# Autodesk Inventor assembly: Ring Stand Clamp
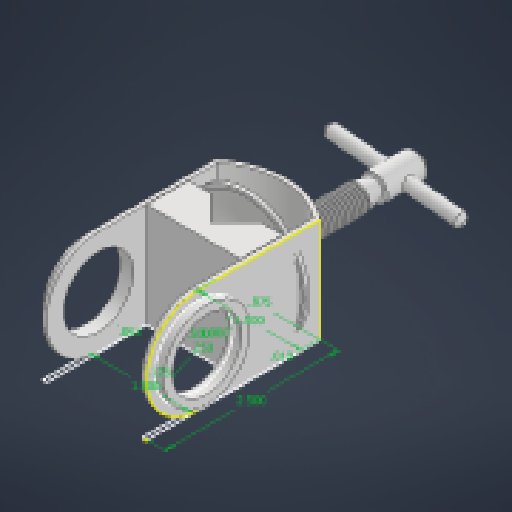
[picture p0: Inventor's stored thumbnail of the model, 512x512]
Saved by Autodesk Inventor 2023.1 (Build 271208000, 208)
## iProperties
Created: 2022-12-06
Part Number: Ring Stand Clamp
Document SubType Name: Assembly
Designer: aubrey-work
Author: aubrey-work
## Documents named in this file (3)
- C:\GitHubRepos\PHYS-12-Website\content\portfolio\FRC Floor Layout\Aubreys\Graduated Shelves\Ring Stand Clamp.iam
- C:\GitHubRepos\PHYS-12-Website\content\portfolio\FRC Floor Layout\Aubreys\Graduated Shelves\Clamp Body.ipt
- C:\GitHubRepos\PHYS-12-Website\content\portfolio\FRC Floor Layout\Aubreys\Graduated Shelves\Clamp Screw.ipt
## Components (2 placed, 2 different names)
1. Clamp Body:1 — Mate:1
2. Clamp Screw:1 — Mate:1
## Relationships (1: Mate 1)
- Mate:1: Clamp Body:1 ↔ Clamp Screw:1
